# Autodesk Inventor assembly: Assembly1
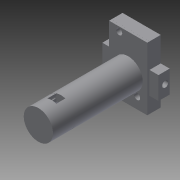
[picture p0: Inventor's stored thumbnail of the model, 180x180]
Saved by Autodesk Inventor 2015 SP1 (Build 190203100, 203)
## iProperties
Created: 2015-06-09
Part Number: Assembly1
Document SubType Name: Assembly
Designer: pc
Author: pc
## Documents named in this file (6)
- C:\Users\pc\Desktop\sensores.diametro\Assembly1.iam
- C:\Users\pc\Desktop\sensores.diametro\soporte.ipt
- C:\Users\pc\Desktop\sensores.diametro\sensores.ipt
- C:\Users\pc\Desktop\sensores.diametro\TORRE.ipt
- C:\Users\pc\Desktop\sensores.diametro\tapa0.2.ipt
- C:\Users\pc\Desktop\sensores.diametro\capuchon.torre.ipt
## Components (5 placed, 5 different names)
1. soporte:1 — Mate:2, Mate:3, Mate:4
2. sensores:1 — Mate:2, Mate:3, Mate:4
3. TORRE:1 — Flush:1, Flush:2, Insert:1
4. tapa0.2:1 — Flush:1, Flush:2
5. capuchon.torre:1 — Insert:1
## Relationships (6: Mate 3, Flush 2, Insert 1)
- Mate:2: soporte:1 ↔ sensores:1
- Mate:3 (0.5 mm): soporte:1 ↔ sensores:1
- Mate:4: soporte:1 ↔ sensores:1
- Flush:1: TORRE:1 ↔ tapa0.2:1
- Flush:2: TORRE:1 ↔ tapa0.2:1
- Insert:1: TORRE:1 ↔ capuchon.torre:1
